# Autodesk Inventor assembly: 1440-01-00 Boite a musique
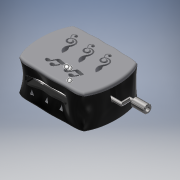
[picture p0: Inventor's stored thumbnail of the model, 180x180]
Saved by Autodesk Inventor 2017 (Build 210142000, 142)
## iProperties
Part Number: 1440-01-00 Boite a musique
Material: Générique
Document SubType Name: Assembly
Designer: Adrien MARY
Author: Adrien MARY
## Documents named in this file (6)
- W:\Professionnel\Conception FABLAB\1440 Boite a musique\1440-01-00 Boite a musique.iam
- W:\Professionnel\Conception FABLAB\1440 Boite a musique\1440-01-01 Couvercle.ipt
- W:\Professionnel\Conception FABLAB\1440 Boite a musique\1440-01-02 Base.ipt
- W:\Professionnel\Conception FABLAB\1440 Boite a musique\Mecanisme\kikkerland-mechanical-music-box-1.snapshot.3\Inventor\Kikkerland Music Box.iam
- W:\Professionnel\Conception FABLAB\1440 Boite a musique\Centre de contenu\fr-FR\ISO 4762(2)\ISO 4762 - M3 x 12ISO.ipt
- W:\Professionnel\Conception FABLAB\1440 Boite a musique\1440-01-04 Bande.ipt
## Components (7 placed, 5 different names)
1. 1440-01-01 Couvercle:1 — Placage:1, Affleurement:4, Affleurement:5
2. 1440-01-02 Base:1 — Placage:1, Affleurement:1, Affleurement:2, Affleurement:3, Logement:1, Placage:2, Logement:2, Logement:3, Logement:4, Affleurement:6
3. Kikkerland Music Box:1 [sub-assembly] — Logement:1, Placage:2, Placage:3, Placage:4
4. ISO 4762 M3 x 12:1 — Logement:3
5. ISO 4762 M3 x 12:2 — Logement:2
6. ISO 4762 M3 x 12:3 — Logement:4
7. 1440-01-04 Bande:1 — Placage:3, Placage:4, Affleurement:7
## Relationships (15: Flush 7, Mate 4, Insert 4)
- Placage:1 [Mate]: 1440-01-01 Couvercle:1 ↔ 1440-01-02 Base:1
- Affleurement:1 [Flush]: 1440-01-02 Base:1
- Affleurement:2 [Flush]: 1440-01-02 Base:1
- Affleurement:3 [Flush]: 1440-01-02 Base:1
- Affleurement:4 [Flush]: 1440-01-01 Couvercle:1
- Affleurement:5 [Flush]: 1440-01-01 Couvercle:1
- Logement:1 [Insert]: 1440-01-02 Base:1 ↔ Kikkerland Music Box:1
- Placage:2 [Mate]: 1440-01-02 Base:1 ↔ Kikkerland Music Box:1
- Logement:2 [Insert]: 1440-01-02 Base:1 ↔ ISO 4762 M3 x 12:2
- Logement:3 [Insert]: 1440-01-02 Base:1 ↔ ISO 4762 M3 x 12:1
- Logement:4 [Insert]: 1440-01-02 Base:1 ↔ ISO 4762 M3 x 12:3
- Placage:3 [Mate]: Kikkerland Music Box:1 ↔ 1440-01-04 Bande:1
- Placage:4 [Mate] (0.5 mm): Kikkerland Music Box:1 ↔ 1440-01-04 Bande:1
- Affleurement:6 [Flush] (-20 mm): 1440-01-02 Base:1
- Affleurement:7 [Flush]: 1440-01-04 Bande:1
